# Autodesk Inventor assembly: testframe
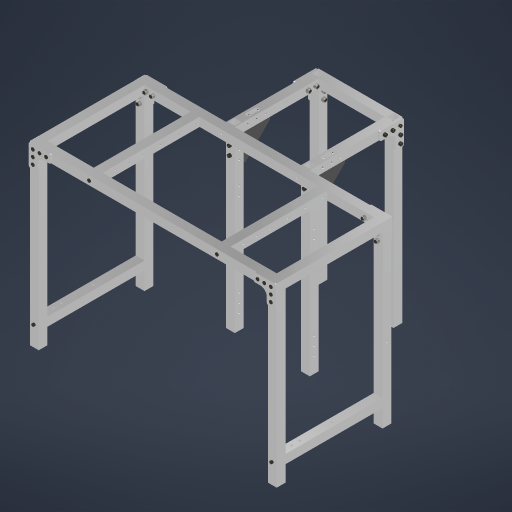
[picture p0: Inventor's stored thumbnail of the model, 512x512]
Saved by Autodesk Inventor 2024.2 (Build 282272000, 272)
## iProperties
Created: 2024-07-23
Part Number: testframe
Document SubType Name: Assembly
Designer: bryan
Mass: 7374.18 g
Surface Area: 16423.9 cm^2
Volume: 2648.19 cm^3
Density: 2.78461 g/cm^3
Author: bryan
## Documents named in this file (28)
- C:\Users\bobsb\OneDrive\Documents\GitHub\1622-2024-Summer-CAD-A-Thon\Structure\STRU_000_StructureAssembly.iam
- C:\Users\bobsb\OneDrive\Documents\GitHub\1622-2024-Summer-CAD-A-Thon\Structure\STRU_001_BilletBlock.ipt
- C:\Users\bobsb\OneDrive\Documents\GitHub\1622-2024-Summer-CAD-A-Thon\Structure\STRU_002_BilletPole_20.56in_Angled.ipt
- C:\Users\bobsb\OneDrive\Documents\GitHub\1622-2024-Summer-CAD-A-Thon\Structure\STRU_003_BilletPole_28in_Angled.ipt
- C:\Users\bobsb\OneDrive\Documents\GitHub\1622-2024-Summer-CAD-A-Thon\Structure\STRU_004_DoubleBillet_90_2.25in.ipt
- C:\Users\bobsb\OneDrive\Documents\GitHub\1622-2024-Summer-CAD-A-Thon\Structure\STRU_007_BilletPole_11in.ipt
- C:\Users\bobsb\OneDrive\Documents\GitHub\1622-2024-Summer-CAD-A-Thon\Structure\STRU_003_BilletPole_28in_Angled_Unique.ipt
- C:\Users\bobsb\OneDrive\Documents\GitHub\1622-2024-Summer-CAD-A-Thon\COTS Library\Fasteners\Bolts\Socket-Head\10-32\COTS_90044A120_Black-Oxide Alloy Steel Socket Head Screw.ipt
- C:\Users\bobsb\OneDrive\Documents\GitHub\1622-2024-Summer-CAD-A-Thon\COTS Library\Fasteners\Bolts\Socket-Head\0.25-20\COTS_90044A123_Black-Oxide Alloy Steel Socket Head Screw.ipt
- C:\Users\bobsb\OneDrive\Documents\GitHub\1622-2024-Summer-CAD-A-Thon\COTS Library\Fasteners\Nuts\COTS_95615A120_Medium-Strength Steel Nylon-Insert Locknut.ipt
- C:\Users\bobsb\OneDrive\Documents\GitHub\1622-2024-Summer-CAD-A-Thon\Structure\STRU_009_FrameBracket_90.ipt
- C:\Users\bobsb\OneDrive\Documents\GitHub\1622-2024-Summer-CAD-A-Thon\Structure\STRU_006_BilletPole_SwerveOffset.ipt
- C:\Users\bobsb\OneDrive\Documents\GitHub\1622-2024-Summer-CAD-A-Thon\Structure\STRU_012_BilletPoleMiddle.ipt
- C:\Users\bobsb\OneDrive\Documents\GitHub\1622-2024-Summer-CAD-A-Thon\Structure\STRU_012_BilletPoleMiddle_Unique.ipt
- C:\Users\bobsb\OneDrive\Documents\GitHub\1622-2024-Summer-CAD-A-Thon\Structure\STRU_014_BilletPole_9in_Angled.ipt
- C:\Users\bobsb\OneDrive\Documents\GitHub\1622-2024-Summer-CAD-A-Thon\Structure\STRU_015_BilletPole_9in.ipt
- C:\Users\bobsb\OneDrive\Documents\GitHub\1622-2024-Summer-CAD-A-Thon\Structure\STRU_016_FrameBracket2_90.ipt
- C:\Users\bobsb\OneDrive\Documents\GitHub\1622-2024-Summer-CAD-A-Thon\Structure\STRU_017_AngleBracket_90_Plastic.ipt
- C:\Users\bobsb\OneDrive\Documents\GitHub\1622-2024-Summer-CAD-A-Thon\COTS Library\Fasteners\Bolts\Socket-Head\0.25-20\COTS_91251A539_Black-Oxide Alloy Steel Socket Head Screw (1).ipt
- C:\Users\bobsb\OneDrive\Documents\GitHub\1622-2024-Summer-CAD-A-Thon\COTS Library\Fasteners\Nuts\COTS_95462A029_Medium-Strength Steel Hex Nut (2).ipt
- C:\Users\bobsb\OneDrive\Documents\GitHub\1622-2024-Summer-CAD-A-Thon\Structure\STRU_019_RubberWasher.ipt
- C:\Users\bobsb\OneDrive\Documents\GitHub\1622-2024-Summer-CAD-A-Thon\Structure\STRU_023_Kenji_11in.ipt
- C:\Users\bobsb\OneDrive\Documents\GitHub\1622-2024-Summer-CAD-A-Thon\Structure\STRU_024_BilletBlock2.ipt
- C:\Users\bobsb\OneDrive\Documents\GitHub\1622-2024-Summer-CAD-A-Thon\COTS Library\Fasteners\Bolts\Socket-Head\0.25-20\COTS_90357A018_Ultra-Low-Profile Socket Head Screw.ipt
- C:\Users\bobsb\OneDrive\Documents\GitHub\1622-2024-Summer-CAD-A-Thon\COTS Library\Fasteners\Bolts\Socket-Head\0.25-20\COTS_90357A021_Ultra-Low-Profile Socket Head Screw.ipt
- C:\Users\bobsb\OneDrive\Documents\GitHub\1622-2024-Summer-CAD-A-Thon\COTS Library\Fasteners\Bolts\Socket-Head\10-32\COTS_91251A352_Black-Oxide Alloy Steel Socket Head.ipt
- C:\Users\bobsb\OneDrive\Documents\GitHub\1622-2024-Summer-CAD-A-Thon\Structure\STRU_026_Bryan_11in.ipt
- C:\Users\bobsb\OneDrive\Documents\GitHub\1622-2024-Summer-CAD-A-Thon\Structure\STRU_000_StructureAssembly\AIP\FEA\err5tqxb5.fres
## Components (137 placed, 26 different names)
1. STRU_001_BilletBlock:2 — Mate:16, Mate:17, Flush:2
2. STRU_002_BilletPole_20.56in_Angled:1 — Mate:1, Mate:4, Mate:5, Mate:41, Mate:53, Mate:54, Flush:10, Mate:91, Mate:92, Mate:127, Mate:147, Mate:148, Mate:470, Mate:471, Flush:63, Mate:527, Mate:528
3. STRU_004_DoubleBillet_90_2.25in:1 — Mate:1, Mate:4, Mate:5, Mate:34, Mate:56, Mate:58, Mate:125, Mate:126
4. STRU_002_BilletPole_20.56in_Angled:2 — Mate:13, Mate:14, Mate:15, Mate:16, Mate:17, Flush:2, Mate:40, Mate:85, Mate:86, Mate:123, Mate:124, Mate:145, Mate:146, Mate:477, Mate:478, Mate:531, Mate:532, Flush:71
5. STRU_004_DoubleBillet_90_2.25in:2 — Mate:13, Mate:14, Mate:15, Mate:36, Mate:57, Mate:100, Mate:121, Mate:122
6. STRU_001_BilletBlock:3 — Mate:185, Mate:186, Flush:26
7. STRU_001_BilletBlock:4 — Mate:180, Mate:181, Flush:25
8. STRU_003_BilletPole_28in_Angled:2 — Mate:47, Flush:8, Flush:9, Mate:55, Mate:118, Mate:130, Mate:153, Mate:154, Mate:155, Mate:156, Mate:178, Mate:182, Mate:484, Mate:485, Mate:486, Mate:490, Flush:68, Mate:491, Mate:492, Mate:493, Mate:541, Flush:73, Mate:542, Mate:543, Mate:544, Mate:545, Flush:74, Mate:548
9. STRU_004_DoubleBillet_90_2.25in:3 — Mate:128, Mate:129, Mate:184
10. STRU_004_DoubleBillet_90_2.25in:4 — Mate:119, Mate:120, Mate:179
11. STRU_001_BilletBlock:5 — Mate:34, Mate:41, Mate:50, Mate:51, Flush:65
12. STRU_001_BilletBlock:8 — Mate:36, Mate:40, Mate:42, Mate:43
13. STRU_007_BilletPole_11in:1 — Flush:9, Mate:50, Mate:51, Mate:55, Mate:59, Mate:537
14. STRU_007_BilletPole_11in:2 — Mate:42, Mate:43, Mate:47, Flush:8, Mate:124
15. STRU_001_BilletBlock:9 — Mate:53, Mate:54, Flush:10
16. STRU_003_BilletPole_28in_Angled_Unique:1 — Mate:56, Mate:57, Mate:58, Mate:59, Mate:83, Mate:84, Mate:93, Mate:94, Mate:98, Mate:149, Mate:150, Mate:151, Mate:152, Mate:159, Mate:160, Mate:164, Mate:165, Flush:28, Mate:221, Flush:29, Mate:223, Flush:68, Mate:559
17. COTS_90044A123_Black-Oxide Alloy Steel Socket Head Screw:6 — Mate:84, Mate:108, Flush:12
18. COTS_90044A123_Black-Oxide Alloy Steel Socket Head Screw:7 — Mate:85, Mate:106, Mate:134, Flush:12, Flush:13, Flush:14
19. COTS_90044A123_Black-Oxide Alloy Steel Socket Head Screw:8 — Mate:83, Mate:107, Flush:13
20. COTS_90044A123_Black-Oxide Alloy Steel Socket Head Screw:9 — Mate:86, Mate:105, Flush:14
21. COTS_90044A123_Black-Oxide Alloy Steel Socket Head Screw:14 — Mate:93, Mate:115, Flush:16
22. COTS_90044A123_Black-Oxide Alloy Steel Socket Head Screw:15 — Mate:92, Mate:114, Flush:17
23. COTS_90044A123_Black-Oxide Alloy Steel Socket Head Screw:16 — Mate:91, Mate:113, Mate:136, Flush:15, Flush:17
24. COTS_90044A123_Black-Oxide Alloy Steel Socket Head Screw:17 — Mate:94, Mate:116, Flush:15, Flush:16
25. COTS_90044A120_Black-Oxide Alloy Steel Socket Head Screw:6 — Mate:100, Mate:135
26. COTS_90044A120_Black-Oxide Alloy Steel Socket Head Screw:7 — Mate:98, Mate:137
27. COTS_95615A120_Medium-Strength Steel Nylon-Insert Locknut:1 — Mate:154, Mate:522
28. COTS_95615A120_Medium-Strength Steel Nylon-Insert Locknut:2 — Mate:153, Mate:521
29. COTS_95615A120_Medium-Strength Steel Nylon-Insert Locknut:3 — Mate:194, Mate:519
30. COTS_95615A120_Medium-Strength Steel Nylon-Insert Locknut:4 — Mate:195, Mate:520
31. COTS_95615A120_Medium-Strength Steel Nylon-Insert Locknut:5 — Mate:107, Mate:152
32. COTS_95615A120_Medium-Strength Steel Nylon-Insert Locknut:6 — Mate:108, Mate:151
33. COTS_95615A120_Medium-Strength Steel Nylon-Insert Locknut:7 — Mate:105, Mate:145
34. COTS_95615A120_Medium-Strength Steel Nylon-Insert Locknut:8 — Mate:106, Mate:146
35. COTS_95615A120_Medium-Strength Steel Nylon-Insert Locknut:9 — Mate:155, Mate:514
36. COTS_95615A120_Medium-Strength Steel Nylon-Insert Locknut:10 — Mate:156, Mate:515
37. COTS_95615A120_Medium-Strength Steel Nylon-Insert Locknut:11 — Mate:189, Mate:513
38. COTS_95615A120_Medium-Strength Steel Nylon-Insert Locknut:12 — Mate:190, Mate:512
39. COTS_95615A120_Medium-Strength Steel Nylon-Insert Locknut:13 — Mate:114, Mate:147
40. COTS_95615A120_Medium-Strength Steel Nylon-Insert Locknut:14 — Mate:113, Mate:148
41. COTS_95615A120_Medium-Strength Steel Nylon-Insert Locknut:15 — Mate:115, Mate:149
42. COTS_95615A120_Medium-Strength Steel Nylon-Insert Locknut:16 — Mate:116, Mate:150
43. STRU_009_FrameBracket_90:1 — Mate:118, Mate:119, Mate:120, Mate:177, Mate:497, Mate:498, Mate:499, Mate:500, Mate:501, Mate:502, Mate:503, Mate:516, Mate:517, Mate:518
44. STRU_009_FrameBracket_90:2 — Mate:125, Mate:126, Mate:127, Mate:136, Mate:137
45. STRU_009_FrameBracket_90:3 — Mate:121, Mate:122, Mate:123, Mate:134, Mate:135
46. STRU_009_FrameBracket_90:4 — Mate:128, Mate:129, Mate:130, Mate:183, Mate:504, Mate:505, Mate:506, Mate:507, Mate:508, Mate:509, Mate:510, Mate:511, Mate:523, Mate:524
47. STRU_001_BilletBlock:11 — Mate:159, Mate:165
48. STRU_001_BilletBlock:12 — Mate:160, Mate:164, Flush:66
49. STRU_006_BilletPole_SwerveOffset:1 — Mate:177, Mate:178, Mate:179, Mate:180, Mate:181, Flush:25, Mate:194, Mate:195, Mate:487, Mate:489, Mate:494, Mate:529, Mate:530, Mate:533
50. STRU_006_BilletPole_SwerveOffset:2 — Mate:182, Mate:183, Mate:184, Mate:185, Mate:186, Flush:26, Mate:189, Mate:190, Mate:475, Mate:488, Mate:495, Mate:525, Mate:526
51. STRU_012_BilletPoleMiddle:6 — Flush:28, Mate:221, Mate:228, Mate:229, Flush:30, Mate:255, Flush:49, Mate:318, Mate:389, Mate:390, Mate:418, Mate:419, Mate:559
52. STRU_012_BilletPoleMiddle:5 — Flush:29, Mate:223, Mate:230, Mate:231, Flush:31, Mate:253, Flush:48, Mate:319, Mate:391, Mate:392, Mate:416, Mate:417
53. STRU_001_BilletBlock:14 — Mate:228, Mate:229, Flush:30
54. STRU_001_BilletBlock:15 — Mate:230, Mate:231, Flush:31
55. STRU_001_BilletBlock:16 — Mate:267, Mate:268, Flush:54
56. STRU_001_BilletBlock:17 — Mate:269, Mate:270, Flush:55
57. STRU_014_BilletPole_9in_Angled:1 — Mate:255, Flush:49, Mate:311, Mate:317, Mate:333, Mate:334, Mate:335, Mate:336, Mate:549, Mate:551, Mate:552, Mate:557, Mate:558
58. STRU_014_BilletPole_9in_Angled:2 — Mate:253, Flush:48, Mate:291, Mate:320, Mate:337, Mate:338, Mate:339, Mate:340, Mate:550, Mate:553, Mate:554, Mate:555, Flush:75, Mate:556
59. STRU_015_BilletPole_9in:1 — Mate:257, Mate:258, Mate:259, Mate:260, Flush:52, Flush:53, Flush:75
60. STRU_001_BilletBlock:18 — Mate:259, Mate:260, Flush:52, Mate:266, Mate:271, Mate:275
61. STRU_001_BilletBlock:19 — Mate:257, Mate:258, Flush:53, Mate:265, Mate:272, Mate:276
62. STRU_012_BilletPoleMiddle_Unique:1 — Mate:265, Mate:267, Mate:268, Flush:54, Mate:272, Mate:277, Mate:278, Mate:279, Mate:304, Mate:316
63. STRU_012_BilletPoleMiddle_Unique:2 — Mate:266, Mate:269, Mate:270, Flush:55, Mate:271, Mate:281, Mate:282, Mate:283, Mate:295, Mate:299
64. COTS_90044A120_Black-Oxide Alloy Steel Socket Head Screw:13 — Mate:275, Mate:284
65. COTS_90044A120_Black-Oxide Alloy Steel Socket Head Screw:14 — Mate:276, Mate:280
66. STRU_016_FrameBracket2_90:1 — Mate:277, Mate:278, Mate:279, Mate:280, Mate:302, Mate:303, Mate:306, Mate:307, Mate:310, Mate:312, Mate:314, Mate:315, Mate:558
67. STRU_016_FrameBracket2_90:2 — Mate:281, Mate:282, Mate:283, Mate:284, Mate:286, Mate:288, Mate:290, Mate:292, Mate:294, Mate:296, Mate:298, Mate:300, Mate:555
68. COTS_90044A123_Black-Oxide Alloy Steel Socket Head Screw:18 — Mate:286, Mate:288, Mate:553
69. COTS_95615A120_Medium-Strength Steel Nylon-Insert Locknut:17 — Mate:556
70. COTS_90044A123_Black-Oxide Alloy Steel Socket Head Screw:19 — Mate:290, Mate:292, Mate:554
71. COTS_95615A120_Medium-Strength Steel Nylon-Insert Locknut:18 — Mate:291
72. COTS_90044A123_Black-Oxide Alloy Steel Socket Head Screw:20 — Mate:294, Mate:296
73. COTS_95615A120_Medium-Strength Steel Nylon-Insert Locknut:19 — Mate:295
74. COTS_90044A123_Black-Oxide Alloy Steel Socket Head Screw:21 — Mate:298, Mate:300
75. COTS_95615A120_Medium-Strength Steel Nylon-Insert Locknut:20 — Mate:299
76. COTS_90044A123_Black-Oxide Alloy Steel Socket Head Screw:22 — Mate:302, Mate:303
77. COTS_95615A120_Medium-Strength Steel Nylon-Insert Locknut:21 — Mate:304
78. COTS_90044A123_Black-Oxide Alloy Steel Socket Head Screw:23 — Mate:306, Mate:307, Mate:551
79. COTS_95615A120_Medium-Strength Steel Nylon-Insert Locknut:22 — Mate:557
80. COTS_90044A123_Black-Oxide Alloy Steel Socket Head Screw:24 — Mate:310, Mate:312, Mate:552
81. COTS_95615A120_Medium-Strength Steel Nylon-Insert Locknut:23 — Mate:311
82. COTS_90044A123_Black-Oxide Alloy Steel Socket Head Screw:25 — Mate:314, Mate:315
83. COTS_95615A120_Medium-Strength Steel Nylon-Insert Locknut:24 — Mate:316
84. STRU_017_AngleBracket_90_Plastic:1 — Mate:317, Mate:318, Mate:453, Mate:454, Mate:458, Mate:462, Mate:463, Mate:467, Mate:549
85. STRU_017_AngleBracket_90_Plastic:2 — Mate:319, Mate:320, Mate:434, Mate:435, Mate:440, Mate:444, Mate:445, Mate:449, Mate:550
86. COTS_91251A539_Black-Oxide Alloy Steel Socket Head Screw (1):1 — Mate:337, Mate:340, Mate:439
87. COTS_91251A539_Black-Oxide Alloy Steel Socket Head Screw (1):2 — Mate:338, Mate:339, Mate:432, Mate:433
88. COTS_91251A539_Black-Oxide Alloy Steel Socket Head Screw (1):4 — Mate:333, Mate:334, Mate:457
89. COTS_91251A539_Black-Oxide Alloy Steel Socket Head Screw (1):5 — Mate:335, Mate:336, Mate:452
90. COTS_90044A123_Black-Oxide Alloy Steel Socket Head Screw:27 — Mate:390, Mate:419, Mate:461
91. COTS_90044A123_Black-Oxide Alloy Steel Socket Head Screw:28 — Mate:389, Mate:418, Mate:466
92. COTS_90044A123_Black-Oxide Alloy Steel Socket Head Screw:29 — Mate:392, Mate:417, Mate:448
93. COTS_90044A123_Black-Oxide Alloy Steel Socket Head Screw:30 — Mate:391, Mate:416, Mate:442, Mate:443
94. COTS_95462A029_Medium-Strength Steel Hex Nut (2):1 — Mate:432, Mate:436
95. STRU_019_RubberWasher:1 — Mate:433, Mate:434, Mate:435, Mate:436, Flush:59
96. COTS_95462A029_Medium-Strength Steel Hex Nut (2):2 — Mate:438, Mate:439
97. STRU_019_RubberWasher:2 — Mate:438, Flush:59, Mate:440
98. COTS_95462A029_Medium-Strength Steel Hex Nut (2):3 — Mate:442
99. STRU_019_RubberWasher:3 — Mate:443, Mate:444, Mate:445, Flush:60
100. COTS_95462A029_Medium-Strength Steel Hex Nut (2):4 — Mate:447, Mate:448
101. STRU_019_RubberWasher:4 — Mate:447, Mate:449, Flush:60
102. COTS_95462A029_Medium-Strength Steel Hex Nut (2):5 — Mate:452
103. STRU_019_RubberWasher:5 — Mate:453, Mate:454, Flush:61
104. COTS_95462A029_Medium-Strength Steel Hex Nut (2):6 — Mate:457
105. STRU_019_RubberWasher:6 — Mate:458, Flush:61
106. COTS_95462A029_Medium-Strength Steel Hex Nut (2):7 — Mate:461
107. STRU_019_RubberWasher:7 — Mate:462, Mate:463, Flush:62
108. COTS_95462A029_Medium-Strength Steel Hex Nut (2):8 — Mate:466
109. STRU_019_RubberWasher:8 — Mate:467, Flush:62
110. STRU_023_Kenji_11in:1 — Mate:472, Mate:473, Flush:63, Mate:475
111. STRU_023_Kenji_11in:2 — Mate:533, Flush:71, Mate:534
112. STRU_001_BilletBlock:22 — Mate:470, Mate:471, Mate:472, Mate:473
113. STRU_001_BilletBlock:23 — Mate:477, Mate:478, Mate:534
114. STRU_024_BilletBlock2:1 — Mate:484, Mate:490, Flush:65, Mate:537
115. STRU_024_BilletBlock2:2 — Mate:487, Flush:69, Mate:492
116. STRU_024_BilletBlock2:3 — Mate:488, Mate:495, Flush:70
117. STRU_024_BilletBlock2:4 — Mate:489, Mate:494, Flush:70
118. STRU_024_BilletBlock2:5 — Mate:486, Flush:67, Flush:69, Mate:491, Mate:539, Mate:540
119. STRU_024_BilletBlock2:6 — Mate:485, Flush:66, Flush:67, Mate:493, Mate:546, Mate:547
120. COTS_90357A018_Ultra-Low-Profile Socket Head Screw:1 — Mate:499, Mate:500, Mate:521
121. COTS_90357A021_Ultra-Low-Profile Socket Head Screw:1 — Mate:497, Mate:498
122. COTS_90357A018_Ultra-Low-Profile Socket Head Screw:2 — Mate:501, Mate:516, Mate:522
123. COTS_90357A018_Ultra-Low-Profile Socket Head Screw:3 — Mate:502, Mate:518, Mate:519
124. COTS_90357A018_Ultra-Low-Profile Socket Head Screw:4 — Mate:503, Mate:517, Mate:520
125. COTS_90357A018_Ultra-Low-Profile Socket Head Screw:5 — Mate:504, Mate:508, Mate:514
126. COTS_90357A018_Ultra-Low-Profile Socket Head Screw:6 — Mate:505, Mate:509, Mate:515
127. COTS_90357A018_Ultra-Low-Profile Socket Head Screw:7 — Mate:506, Mate:510, Mate:513
128. COTS_90357A018_Ultra-Low-Profile Socket Head Screw:8 — Mate:507, Mate:511, Mate:512
129. COTS_90357A021_Ultra-Low-Profile Socket Head Screw:2 — Mate:523, Mate:524
130. COTS_91251A352_Black-Oxide Alloy Steel Socket Head:1 — Mate:525, Mate:526
131. COTS_91251A352_Black-Oxide Alloy Steel Socket Head:2 — Mate:527, Mate:528
132. COTS_91251A352_Black-Oxide Alloy Steel Socket Head:3 — Mate:529, Mate:530
133. COTS_91251A352_Black-Oxide Alloy Steel Socket Head:4 — Mate:531, Mate:532
134. STRU_026_Bryan_11in:2 — Mate:539, Mate:540, Mate:541, Flush:73
135. COTS_90357A021_Ultra-Low-Profile Socket Head Screw:3 — Mate:542, Mate:543
136. COTS_90357A021_Ultra-Low-Profile Socket Head Screw:4 — Mate:544, Mate:545
137. STRU_026_Bryan_11in:3 — Mate:546, Mate:547, Flush:74, Mate:548
## Relationships (327: Mate 290, Flush 37)
- Mate:1: STRU_002_BilletPole_20.56in_Angled:1 ↔ STRU_004_DoubleBillet_90_2.25in:1
- Mate:4: STRU_002_BilletPole_20.56in_Angled:1 ↔ STRU_004_DoubleBillet_90_2.25in:1
- Mate:5: STRU_002_BilletPole_20.56in_Angled:1 ↔ STRU_004_DoubleBillet_90_2.25in:1
- Mate:13: STRU_002_BilletPole_20.56in_Angled:2 ↔ STRU_004_DoubleBillet_90_2.25in:2
- Mate:14: STRU_002_BilletPole_20.56in_Angled:2 ↔ STRU_004_DoubleBillet_90_2.25in:2
- Mate:15: STRU_002_BilletPole_20.56in_Angled:2 ↔ STRU_004_DoubleBillet_90_2.25in:2
- Mate:16: STRU_001_BilletBlock:2 ↔ STRU_002_BilletPole_20.56in_Angled:2
- Mate:17: STRU_001_BilletBlock:2 ↔ STRU_002_BilletPole_20.56in_Angled:2
- Flush:2: STRU_001_BilletBlock:2 ↔ STRU_002_BilletPole_20.56in_Angled:2
- [Mate]: STRU_003_BilletPole_28in_Angled:2 ↔ STRU_004_DoubleBillet_90_2.25in:3
- [Mate]: STRU_003_BilletPole_28in_Angled:2 ↔ STRU_004_DoubleBillet_90_2.25in:3
- [Mate]: STRU_003_BilletPole_28in_Angled:2 ↔ STRU_004_DoubleBillet_90_2.25in:3
- [Mate]: STRU_003_BilletPole_28in_Angled:2 ↔ STRU_004_DoubleBillet_90_2.25in:4
- [Mate]: STRU_003_BilletPole_28in_Angled:2 ↔ STRU_004_DoubleBillet_90_2.25in:4
- [Mate]: STRU_003_BilletPole_28in_Angled:2 ↔ STRU_004_DoubleBillet_90_2.25in:4
- Mate:34: STRU_004_DoubleBillet_90_2.25in:1 ↔ STRU_001_BilletBlock:5
- Mate:36: STRU_004_DoubleBillet_90_2.25in:2 ↔ STRU_001_BilletBlock:8
- Mate:40: STRU_002_BilletPole_20.56in_Angled:2 ↔ STRU_001_BilletBlock:8
- Mate:41: STRU_002_BilletPole_20.56in_Angled:1 ↔ STRU_001_BilletBlock:5
- Mate:42: STRU_001_BilletBlock:8 ↔ STRU_007_BilletPole_11in:2
- Mate:43: STRU_001_BilletBlock:8 ↔ STRU_007_BilletPole_11in:2
- Mate:47: STRU_003_BilletPole_28in_Angled:2 ↔ STRU_007_BilletPole_11in:2
- Flush:8: STRU_003_BilletPole_28in_Angled:2 ↔ STRU_007_BilletPole_11in:2
- Flush:9: STRU_003_BilletPole_28in_Angled:2 ↔ STRU_007_BilletPole_11in:1
- Mate:50: STRU_001_BilletBlock:5 ↔ STRU_007_BilletPole_11in:1
- Mate:51: STRU_001_BilletBlock:5 ↔ STRU_007_BilletPole_11in:1
- Mate:53: STRU_002_BilletPole_20.56in_Angled:1 ↔ STRU_001_BilletBlock:9
- Mate:54: STRU_002_BilletPole_20.56in_Angled:1 ↔ STRU_001_BilletBlock:9
- Flush:10: STRU_002_BilletPole_20.56in_Angled:1 ↔ STRU_001_BilletBlock:9
- Mate:55: STRU_003_BilletPole_28in_Angled:2 ↔ STRU_007_BilletPole_11in:1
- Mate:56: STRU_004_DoubleBillet_90_2.25in:1 ↔ STRU_003_BilletPole_28in_Angled_Unique:1
- Mate:57: STRU_004_DoubleBillet_90_2.25in:2 ↔ STRU_003_BilletPole_28in_Angled_Unique:1
- Mate:58: STRU_004_DoubleBillet_90_2.25in:1 ↔ STRU_003_BilletPole_28in_Angled_Unique:1
- Mate:59: STRU_007_BilletPole_11in:1 ↔ STRU_003_BilletPole_28in_Angled_Unique:1
- Mate:83: STRU_003_BilletPole_28in_Angled_Unique:1 ↔ COTS_90044A123_Black-Oxide Alloy Steel Socket Head Screw:8
- Mate:84: STRU_003_BilletPole_28in_Angled_Unique:1 ↔ COTS_90044A123_Black-Oxide Alloy Steel Socket Head Screw:6
- Mate:85: STRU_002_BilletPole_20.56in_Angled:2 ↔ COTS_90044A123_Black-Oxide Alloy Steel Socket Head Screw:7
- Mate:86: STRU_002_BilletPole_20.56in_Angled:2 ↔ COTS_90044A123_Black-Oxide Alloy Steel Socket Head Screw:9
- Mate:91: STRU_002_BilletPole_20.56in_Angled:1 ↔ COTS_90044A123_Black-Oxide Alloy Steel Socket Head Screw:16
- Mate:92: STRU_002_BilletPole_20.56in_Angled:1 ↔ COTS_90044A123_Black-Oxide Alloy Steel Socket Head Screw:15
- Mate:93: STRU_003_BilletPole_28in_Angled_Unique:1 ↔ COTS_90044A123_Black-Oxide Alloy Steel Socket Head Screw:14
- Mate:94: STRU_003_BilletPole_28in_Angled_Unique:1 ↔ COTS_90044A123_Black-Oxide Alloy Steel Socket Head Screw:17
- Mate:98: STRU_003_BilletPole_28in_Angled_Unique:1 ↔ COTS_90044A120_Black-Oxide Alloy Steel Socket Head Screw:7
- Mate:100: STRU_004_DoubleBillet_90_2.25in:2 ↔ COTS_90044A120_Black-Oxide Alloy Steel Socket Head Screw:6
- Mate:105: COTS_90044A123_Black-Oxide Alloy Steel Socket Head Screw:9 ↔ COTS_95615A120_Medium-Strength Steel Nylon-Insert Locknut:7
- Mate:106: COTS_90044A123_Black-Oxide Alloy Steel Socket Head Screw:7 ↔ COTS_95615A120_Medium-Strength Steel Nylon-Insert Locknut:8
- Mate:107: COTS_90044A123_Black-Oxide Alloy Steel Socket Head Screw:8 ↔ COTS_95615A120_Medium-Strength Steel Nylon-Insert Locknut:5
- Mate:108: COTS_90044A123_Black-Oxide Alloy Steel Socket Head Screw:6 ↔ COTS_95615A120_Medium-Strength Steel Nylon-Insert Locknut:6
- Mate:113: COTS_90044A123_Black-Oxide Alloy Steel Socket Head Screw:16 ↔ COTS_95615A120_Medium-Strength Steel Nylon-Insert Locknut:14
- Mate:114: COTS_90044A123_Black-Oxide Alloy Steel Socket Head Screw:15 ↔ COTS_95615A120_Medium-Strength Steel Nylon-Insert Locknut:13
- Mate:115: COTS_90044A123_Black-Oxide Alloy Steel Socket Head Screw:14 ↔ COTS_95615A120_Medium-Strength Steel Nylon-Insert Locknut:15
- Mate:116: COTS_90044A123_Black-Oxide Alloy Steel Socket Head Screw:17 ↔ COTS_95615A120_Medium-Strength Steel Nylon-Insert Locknut:16
- Mate:118: STRU_003_BilletPole_28in_Angled:2 ↔ STRU_009_FrameBracket_90:1
- Mate:119: STRU_004_DoubleBillet_90_2.25in:4 ↔ STRU_009_FrameBracket_90:1
- Mate:120: STRU_004_DoubleBillet_90_2.25in:4 ↔ STRU_009_FrameBracket_90:1
- Mate:121: STRU_004_DoubleBillet_90_2.25in:2 ↔ STRU_009_FrameBracket_90:3
- Mate:122: STRU_004_DoubleBillet_90_2.25in:2 ↔ STRU_009_FrameBracket_90:3
- Mate:123: STRU_002_BilletPole_20.56in_Angled:2 ↔ STRU_009_FrameBracket_90:3
- Mate:124: STRU_002_BilletPole_20.56in_Angled:2 ↔ STRU_007_BilletPole_11in:2
- Mate:125: STRU_004_DoubleBillet_90_2.25in:1 ↔ STRU_009_FrameBracket_90:2
- Mate:126: STRU_004_DoubleBillet_90_2.25in:1 ↔ STRU_009_FrameBracket_90:2
- Mate:127: STRU_002_BilletPole_20.56in_Angled:1 ↔ STRU_009_FrameBracket_90:2
- Mate:128: STRU_004_DoubleBillet_90_2.25in:3 ↔ STRU_009_FrameBracket_90:4
- Mate:129: STRU_004_DoubleBillet_90_2.25in:3 ↔ STRU_009_FrameBracket_90:4
- Mate:130: STRU_003_BilletPole_28in_Angled:2 ↔ STRU_009_FrameBracket_90:4
- Mate:134: COTS_90044A123_Black-Oxide Alloy Steel Socket Head Screw:7 ↔ STRU_009_FrameBracket_90:3
- Flush:12: COTS_90044A123_Black-Oxide Alloy Steel Socket Head Screw:6 ↔ COTS_90044A123_Black-Oxide Alloy Steel Socket Head Screw:7
- Mate:135: COTS_90044A120_Black-Oxide Alloy Steel Socket Head Screw:6 ↔ STRU_009_FrameBracket_90:3
- Flush:13: COTS_90044A123_Black-Oxide Alloy Steel Socket Head Screw:7 ↔ COTS_90044A123_Black-Oxide Alloy Steel Socket Head Screw:8
- Flush:14: COTS_90044A123_Black-Oxide Alloy Steel Socket Head Screw:7 ↔ COTS_90044A123_Black-Oxide Alloy Steel Socket Head Screw:9
- Mate:136: COTS_90044A123_Black-Oxide Alloy Steel Socket Head Screw:16 ↔ STRU_009_FrameBracket_90:2
- Mate:137: COTS_90044A120_Black-Oxide Alloy Steel Socket Head Screw:7 ↔ STRU_009_FrameBracket_90:2
- Flush:15: COTS_90044A123_Black-Oxide Alloy Steel Socket Head Screw:16 ↔ COTS_90044A123_Black-Oxide Alloy Steel Socket Head Screw:17
- Flush:16: COTS_90044A123_Black-Oxide Alloy Steel Socket Head Screw:14 ↔ COTS_90044A123_Black-Oxide Alloy Steel Socket Head Screw:17
- Flush:17: COTS_90044A123_Black-Oxide Alloy Steel Socket Head Screw:15 ↔ COTS_90044A123_Black-Oxide Alloy Steel Socket Head Screw:16
- Mate:145: STRU_002_BilletPole_20.56in_Angled:2 ↔ COTS_95615A120_Medium-Strength Steel Nylon-Insert Locknut:7
- Mate:146: STRU_002_BilletPole_20.56in_Angled:2 ↔ COTS_95615A120_Medium-Strength Steel Nylon-Insert Locknut:8
- Mate:147: STRU_002_BilletPole_20.56in_Angled:1 ↔ COTS_95615A120_Medium-Strength Steel Nylon-Insert Locknut:13
- Mate:148: STRU_002_BilletPole_20.56in_Angled:1 ↔ COTS_95615A120_Medium-Strength Steel Nylon-Insert Locknut:14
- Mate:149: STRU_003_BilletPole_28in_Angled_Unique:1 ↔ COTS_95615A120_Medium-Strength Steel Nylon-Insert Locknut:15
- Mate:150: STRU_003_BilletPole_28in_Angled_Unique:1 ↔ COTS_95615A120_Medium-Strength Steel Nylon-Insert Locknut:16
- Mate:151: STRU_003_BilletPole_28in_Angled_Unique:1 ↔ COTS_95615A120_Medium-Strength Steel Nylon-Insert Locknut:6
- Mate:152: STRU_003_BilletPole_28in_Angled_Unique:1 ↔ COTS_95615A120_Medium-Strength Steel Nylon-Insert Locknut:5
- Mate:153: STRU_003_BilletPole_28in_Angled:2 ↔ COTS_95615A120_Medium-Strength Steel Nylon-Insert Locknut:2
- Mate:154: STRU_003_BilletPole_28in_Angled:2 ↔ COTS_95615A120_Medium-Strength Steel Nylon-Insert Locknut:1
- Mate:155: STRU_003_BilletPole_28in_Angled:2 ↔ COTS_95615A120_Medium-Strength Steel Nylon-Insert Locknut:9
- Mate:156: STRU_003_BilletPole_28in_Angled:2 ↔ COTS_95615A120_Medium-Strength Steel Nylon-Insert Locknut:10
- Mate:159: STRU_003_BilletPole_28in_Angled_Unique:1 ↔ STRU_001_BilletBlock:11
- Mate:160: STRU_003_BilletPole_28in_Angled_Unique:1 ↔ STRU_001_BilletBlock:12
- Mate:164: STRU_003_BilletPole_28in_Angled_Unique:1 ↔ STRU_001_BilletBlock:12
- Mate:165: STRU_003_BilletPole_28in_Angled_Unique:1 ↔ STRU_001_BilletBlock:11
- Mate:177: STRU_009_FrameBracket_90:1 ↔ STRU_006_BilletPole_SwerveOffset:1
- Mate:178: STRU_003_BilletPole_28in_Angled:2 ↔ STRU_006_BilletPole_SwerveOffset:1
- Mate:179: STRU_004_DoubleBillet_90_2.25in:4 ↔ STRU_006_BilletPole_SwerveOffset:1
- Mate:180: STRU_001_BilletBlock:4 ↔ STRU_006_BilletPole_SwerveOffset:1
- Mate:181: STRU_001_BilletBlock:4 ↔ STRU_006_BilletPole_SwerveOffset:1
- Flush:25: STRU_001_BilletBlock:4 ↔ STRU_006_BilletPole_SwerveOffset:1
- Mate:182: STRU_003_BilletPole_28in_Angled:2 ↔ STRU_006_BilletPole_SwerveOffset:2
- Mate:183: STRU_009_FrameBracket_90:4 ↔ STRU_006_BilletPole_SwerveOffset:2
- Mate:184: STRU_004_DoubleBillet_90_2.25in:3 ↔ STRU_006_BilletPole_SwerveOffset:2
- Mate:185: STRU_001_BilletBlock:3 ↔ STRU_006_BilletPole_SwerveOffset:2
- Mate:186: STRU_001_BilletBlock:3 ↔ STRU_006_BilletPole_SwerveOffset:2
- Flush:26: STRU_001_BilletBlock:3 ↔ STRU_006_BilletPole_SwerveOffset:2
- Mate:189: COTS_95615A120_Medium-Strength Steel Nylon-Insert Locknut:11 ↔ STRU_006_BilletPole_SwerveOffset:2
- Mate:190: COTS_95615A120_Medium-Strength Steel Nylon-Insert Locknut:12 ↔ STRU_006_BilletPole_SwerveOffset:2
- Mate:194: COTS_95615A120_Medium-Strength Steel Nylon-Insert Locknut:3 ↔ STRU_006_BilletPole_SwerveOffset:1
- Mate:195: COTS_95615A120_Medium-Strength Steel Nylon-Insert Locknut:4 ↔ STRU_006_BilletPole_SwerveOffset:1
- Flush:28: STRU_003_BilletPole_28in_Angled_Unique:1 ↔ STRU_012_BilletPoleMiddle:6
- Mate:221: STRU_003_BilletPole_28in_Angled_Unique:1 ↔ STRU_012_BilletPoleMiddle:6
- Flush:29: STRU_003_BilletPole_28in_Angled_Unique:1 ↔ STRU_012_BilletPoleMiddle:5
- Mate:223: STRU_003_BilletPole_28in_Angled_Unique:1 ↔ STRU_012_BilletPoleMiddle:5
- Mate:228: STRU_012_BilletPoleMiddle:6 ↔ STRU_001_BilletBlock:14
- Mate:229: STRU_012_BilletPoleMiddle:6 ↔ STRU_001_BilletBlock:14
- Flush:30: STRU_012_BilletPoleMiddle:6 ↔ STRU_001_BilletBlock:14
- Mate:230: STRU_012_BilletPoleMiddle:5 ↔ STRU_001_BilletBlock:15
- Mate:231: STRU_012_BilletPoleMiddle:5 ↔ STRU_001_BilletBlock:15
- Flush:31: STRU_012_BilletPoleMiddle:5 ↔ STRU_001_BilletBlock:15
- Mate:253: STRU_012_BilletPoleMiddle:5 ↔ STRU_014_BilletPole_9in_Angled:2
- Flush:48: STRU_012_BilletPoleMiddle:5 ↔ STRU_014_BilletPole_9in_Angled:2
- Mate:255: STRU_012_BilletPoleMiddle:6 ↔ STRU_014_BilletPole_9in_Angled:1
- Flush:49: STRU_012_BilletPoleMiddle:6 ↔ STRU_014_BilletPole_9in_Angled:1
- Mate:257: STRU_015_BilletPole_9in:1 ↔ STRU_001_BilletBlock:19
- Mate:258: STRU_015_BilletPole_9in:1 ↔ STRU_001_BilletBlock:19
- Mate:259: STRU_015_BilletPole_9in:1 ↔ STRU_001_BilletBlock:18
- Mate:260: STRU_015_BilletPole_9in:1 ↔ STRU_001_BilletBlock:18
- Flush:52: STRU_015_BilletPole_9in:1 ↔ STRU_001_BilletBlock:18
- Flush:53: STRU_015_BilletPole_9in:1 ↔ STRU_001_BilletBlock:19
- Mate:265: STRU_001_BilletBlock:19 ↔ STRU_012_BilletPoleMiddle_Unique:1
- Mate:266: STRU_001_BilletBlock:18 ↔ STRU_012_BilletPoleMiddle_Unique:2
- Mate:267: STRU_001_BilletBlock:16 ↔ STRU_012_BilletPoleMiddle_Unique:1
- Mate:268: STRU_001_BilletBlock:16 ↔ STRU_012_BilletPoleMiddle_Unique:1
- Flush:54: STRU_001_BilletBlock:16 ↔ STRU_012_BilletPoleMiddle_Unique:1
- Mate:269: STRU_001_BilletBlock:17 ↔ STRU_012_BilletPoleMiddle_Unique:2
- Mate:270: STRU_001_BilletBlock:17 ↔ STRU_012_BilletPoleMiddle_Unique:2
- Flush:55: STRU_001_BilletBlock:17 ↔ STRU_012_BilletPoleMiddle_Unique:2
- Mate:271: STRU_001_BilletBlock:18 ↔ STRU_012_BilletPoleMiddle_Unique:2
- Mate:272: STRU_001_BilletBlock:19 ↔ STRU_012_BilletPoleMiddle_Unique:1
- Mate:275: STRU_001_BilletBlock:18 ↔ COTS_90044A120_Black-Oxide Alloy Steel Socket Head Screw:13
- Mate:276: STRU_001_BilletBlock:19 ↔ COTS_90044A120_Black-Oxide Alloy Steel Socket Head Screw:14
- Mate:277: STRU_012_BilletPoleMiddle_Unique:1 ↔ STRU_016_FrameBracket2_90:1
- Mate:278: STRU_012_BilletPoleMiddle_Unique:1 ↔ STRU_016_FrameBracket2_90:1
- Mate:279: STRU_012_BilletPoleMiddle_Unique:1 ↔ STRU_016_FrameBracket2_90:1
- Mate:280: COTS_90044A120_Black-Oxide Alloy Steel Socket Head Screw:14 ↔ STRU_016_FrameBracket2_90:1
- Mate:281: STRU_012_BilletPoleMiddle_Unique:2 ↔ STRU_016_FrameBracket2_90:2
- Mate:282: STRU_012_BilletPoleMiddle_Unique:2 ↔ STRU_016_FrameBracket2_90:2
- Mate:283: STRU_012_BilletPoleMiddle_Unique:2 ↔ STRU_016_FrameBracket2_90:2
- Mate:284: COTS_90044A120_Black-Oxide Alloy Steel Socket Head Screw:13 ↔ STRU_016_FrameBracket2_90:2
- [Mate]: COTS_90044A123_Black-Oxide Alloy Steel Socket Head Screw:18 ↔ COTS_95615A120_Medium-Strength Steel Nylon-Insert Locknut:17
- Mate:286: STRU_016_FrameBracket2_90:2 ↔ COTS_90044A123_Black-Oxide Alloy Steel Socket Head Screw:18
- Mate:288: STRU_016_FrameBracket2_90:2 ↔ COTS_90044A123_Black-Oxide Alloy Steel Socket Head Screw:18
- [Mate]: COTS_90044A123_Black-Oxide Alloy Steel Socket Head Screw:19 ↔ COTS_95615A120_Medium-Strength Steel Nylon-Insert Locknut:18
- Mate:290: STRU_016_FrameBracket2_90:2 ↔ COTS_90044A123_Black-Oxide Alloy Steel Socket Head Screw:19
- Mate:291: STRU_014_BilletPole_9in_Angled:2 ↔ COTS_95615A120_Medium-Strength Steel Nylon-Insert Locknut:18
- Mate:292: STRU_016_FrameBracket2_90:2 ↔ COTS_90044A123_Black-Oxide Alloy Steel Socket Head Screw:19
- [Mate]: COTS_90044A123_Black-Oxide Alloy Steel Socket Head Screw:20 ↔ COTS_95615A120_Medium-Strength Steel Nylon-Insert Locknut:19
- Mate:294: STRU_016_FrameBracket2_90:2 ↔ COTS_90044A123_Black-Oxide Alloy Steel Socket Head Screw:20
- Mate:295: STRU_012_BilletPoleMiddle_Unique:2 ↔ COTS_95615A120_Medium-Strength Steel Nylon-Insert Locknut:19
- Mate:296: STRU_016_FrameBracket2_90:2 ↔ COTS_90044A123_Black-Oxide Alloy Steel Socket Head Screw:20
- [Mate]: COTS_90044A123_Black-Oxide Alloy Steel Socket Head Screw:21 ↔ COTS_95615A120_Medium-Strength Steel Nylon-Insert Locknut:20
- Mate:298: STRU_016_FrameBracket2_90:2 ↔ COTS_90044A123_Black-Oxide Alloy Steel Socket Head Screw:21
- Mate:299: STRU_012_BilletPoleMiddle_Unique:2 ↔ COTS_95615A120_Medium-Strength Steel Nylon-Insert Locknut:20
- Mate:300: STRU_016_FrameBracket2_90:2 ↔ COTS_90044A123_Black-Oxide Alloy Steel Socket Head Screw:21
- [Mate]: COTS_90044A123_Black-Oxide Alloy Steel Socket Head Screw:22 ↔ COTS_95615A120_Medium-Strength Steel Nylon-Insert Locknut:21
- Mate:302: STRU_016_FrameBracket2_90:1 ↔ COTS_90044A123_Black-Oxide Alloy Steel Socket Head Screw:22
- Mate:303: STRU_016_FrameBracket2_90:1 ↔ COTS_90044A123_Black-Oxide Alloy Steel Socket Head Screw:22
- Mate:304: STRU_012_BilletPoleMiddle_Unique:1 ↔ COTS_95615A120_Medium-Strength Steel Nylon-Insert Locknut:21
- [Mate]: COTS_90044A123_Black-Oxide Alloy Steel Socket Head Screw:23 ↔ COTS_95615A120_Medium-Strength Steel Nylon-Insert Locknut:22
- Mate:306: STRU_016_FrameBracket2_90:1 ↔ COTS_90044A123_Black-Oxide Alloy Steel Socket Head Screw:23
- Mate:307: STRU_016_FrameBracket2_90:1 ↔ COTS_90044A123_Black-Oxide Alloy Steel Socket Head Screw:23
- [Mate]: COTS_90044A123_Black-Oxide Alloy Steel Socket Head Screw:24 ↔ COTS_95615A120_Medium-Strength Steel Nylon-Insert Locknut:23
- Mate:310: STRU_016_FrameBracket2_90:1 ↔ COTS_90044A123_Black-Oxide Alloy Steel Socket Head Screw:24
- Mate:311: STRU_014_BilletPole_9in_Angled:1 ↔ COTS_95615A120_Medium-Strength Steel Nylon-Insert Locknut:23
- Mate:312: STRU_016_FrameBracket2_90:1 ↔ COTS_90044A123_Black-Oxide Alloy Steel Socket Head Screw:24
- [Mate]: COTS_90044A123_Black-Oxide Alloy Steel Socket Head Screw:25 ↔ COTS_95615A120_Medium-Strength Steel Nylon-Insert Locknut:24
- Mate:314: STRU_016_FrameBracket2_90:1 ↔ COTS_90044A123_Black-Oxide Alloy Steel Socket Head Screw:25
- Mate:315: STRU_016_FrameBracket2_90:1 ↔ COTS_90044A123_Black-Oxide Alloy Steel Socket Head Screw:25
- Mate:316: STRU_012_BilletPoleMiddle_Unique:1 ↔ COTS_95615A120_Medium-Strength Steel Nylon-Insert Locknut:24
- Mate:317: STRU_014_BilletPole_9in_Angled:1 ↔ STRU_017_AngleBracket_90_Plastic:1
- Mate:318: STRU_012_BilletPoleMiddle:6 ↔ STRU_017_AngleBracket_90_Plastic:1
- Mate:319: STRU_012_BilletPoleMiddle:5 ↔ STRU_017_AngleBracket_90_Plastic:2
- Mate:320: STRU_014_BilletPole_9in_Angled:2 ↔ STRU_017_AngleBracket_90_Plastic:2
- Mate:333: STRU_014_BilletPole_9in_Angled:1 ↔ COTS_91251A539_Black-Oxide Alloy Steel Socket Head Screw (1):4
- Mate:334: STRU_014_BilletPole_9in_Angled:1 ↔ COTS_91251A539_Black-Oxide Alloy Steel Socket Head Screw (1):4
- Mate:335: STRU_014_BilletPole_9in_Angled:1 ↔ COTS_91251A539_Black-Oxide Alloy Steel Socket Head Screw (1):5
- Mate:336: STRU_014_BilletPole_9in_Angled:1 ↔ COTS_91251A539_Black-Oxide Alloy Steel Socket Head Screw (1):5
- Mate:337: STRU_014_BilletPole_9in_Angled:2 ↔ COTS_91251A539_Black-Oxide Alloy Steel Socket Head Screw (1):1
- Mate:338: STRU_014_BilletPole_9in_Angled:2 ↔ COTS_91251A539_Black-Oxide Alloy Steel Socket Head Screw (1):2
- Mate:339: STRU_014_BilletPole_9in_Angled:2 ↔ COTS_91251A539_Black-Oxide Alloy Steel Socket Head Screw (1):2
- Mate:340: STRU_014_BilletPole_9in_Angled:2 ↔ COTS_91251A539_Black-Oxide Alloy Steel Socket Head Screw (1):1
- Mate:389: STRU_012_BilletPoleMiddle:6 ↔ COTS_90044A123_Black-Oxide Alloy Steel Socket Head Screw:28
- Mate:390: STRU_012_BilletPoleMiddle:6 ↔ COTS_90044A123_Black-Oxide Alloy Steel Socket Head Screw:27
- Mate:391: STRU_012_BilletPoleMiddle:5 ↔ COTS_90044A123_Black-Oxide Alloy Steel Socket Head Screw:30
- Mate:392: STRU_012_BilletPoleMiddle:5 ↔ COTS_90044A123_Black-Oxide Alloy Steel Socket Head Screw:29
- Mate:416: STRU_012_BilletPoleMiddle:5 ↔ COTS_90044A123_Black-Oxide Alloy Steel Socket Head Screw:30
- Mate:417: STRU_012_BilletPoleMiddle:5 ↔ COTS_90044A123_Black-Oxide Alloy Steel Socket Head Screw:29
- Mate:418: STRU_012_BilletPoleMiddle:6 ↔ COTS_90044A123_Black-Oxide Alloy Steel Socket Head Screw:28
- Mate:419: STRU_012_BilletPoleMiddle:6 ↔ COTS_90044A123_Black-Oxide Alloy Steel Socket Head Screw:27
- Mate:432: COTS_91251A539_Black-Oxide Alloy Steel Socket Head Screw (1):2 ↔ COTS_95462A029_Medium-Strength Steel Hex Nut (2):1
- Mate:433: COTS_91251A539_Black-Oxide Alloy Steel Socket Head Screw (1):2 ↔ STRU_019_RubberWasher:1
- Mate:434: STRU_017_AngleBracket_90_Plastic:2 ↔ STRU_019_RubberWasher:1
- Mate:435: STRU_017_AngleBracket_90_Plastic:2 ↔ STRU_019_RubberWasher:1
- Mate:436: COTS_95462A029_Medium-Strength Steel Hex Nut (2):1 ↔ STRU_019_RubberWasher:1
- [Mate]: COTS_95462A029_Medium-Strength Steel Hex Nut (2):2 ↔ STRU_019_RubberWasher:2
- Mate:438: COTS_95462A029_Medium-Strength Steel Hex Nut (2):2 ↔ STRU_019_RubberWasher:2
- Mate:439: COTS_91251A539_Black-Oxide Alloy Steel Socket Head Screw (1):1 ↔ COTS_95462A029_Medium-Strength Steel Hex Nut (2):2
- Flush:59: STRU_019_RubberWasher:1 ↔ STRU_019_RubberWasher:2
- Mate:440: STRU_017_AngleBracket_90_Plastic:2 ↔ STRU_019_RubberWasher:2
- [Mate]: COTS_95462A029_Medium-Strength Steel Hex Nut (2):3 ↔ STRU_019_RubberWasher:3
- Mate:442: COTS_90044A123_Black-Oxide Alloy Steel Socket Head Screw:30 ↔ COTS_95462A029_Medium-Strength Steel Hex Nut (2):3
- Mate:443: COTS_90044A123_Black-Oxide Alloy Steel Socket Head Screw:30 ↔ STRU_019_RubberWasher:3
- Mate:444: STRU_017_AngleBracket_90_Plastic:2 ↔ STRU_019_RubberWasher:3
- Mate:445: STRU_017_AngleBracket_90_Plastic:2 ↔ STRU_019_RubberWasher:3
- [Mate]: COTS_95462A029_Medium-Strength Steel Hex Nut (2):4 ↔ STRU_019_RubberWasher:4
- Mate:447: COTS_95462A029_Medium-Strength Steel Hex Nut (2):4 ↔ STRU_019_RubberWasher:4
- Mate:448: COTS_90044A123_Black-Oxide Alloy Steel Socket Head Screw:29 ↔ COTS_95462A029_Medium-Strength Steel Hex Nut (2):4
- Mate:449: STRU_017_AngleBracket_90_Plastic:2 ↔ STRU_019_RubberWasher:4
- Flush:60: STRU_019_RubberWasher:3 ↔ STRU_019_RubberWasher:4
- [Mate]: COTS_95462A029_Medium-Strength Steel Hex Nut (2):5 ↔ STRU_019_RubberWasher:5
- [Mate]: COTS_95462A029_Medium-Strength Steel Hex Nut (2):5 ↔ STRU_019_RubberWasher:5
- Mate:452: COTS_91251A539_Black-Oxide Alloy Steel Socket Head Screw (1):5 ↔ COTS_95462A029_Medium-Strength Steel Hex Nut (2):5
- Mate:453: STRU_017_AngleBracket_90_Plastic:1 ↔ STRU_019_RubberWasher:5
- Mate:454: STRU_017_AngleBracket_90_Plastic:1 ↔ STRU_019_RubberWasher:5
- [Mate]: COTS_95462A029_Medium-Strength Steel Hex Nut (2):6 ↔ STRU_019_RubberWasher:6
- [Mate]: COTS_95462A029_Medium-Strength Steel Hex Nut (2):6 ↔ STRU_019_RubberWasher:6
- Mate:457: COTS_91251A539_Black-Oxide Alloy Steel Socket Head Screw (1):4 ↔ COTS_95462A029_Medium-Strength Steel Hex Nut (2):6
- Mate:458: STRU_017_AngleBracket_90_Plastic:1 ↔ STRU_019_RubberWasher:6
- Flush:61: STRU_019_RubberWasher:5 ↔ STRU_019_RubberWasher:6
- [Mate]: COTS_95462A029_Medium-Strength Steel Hex Nut (2):7 ↔ STRU_019_RubberWasher:7
- [Mate]: COTS_95462A029_Medium-Strength Steel Hex Nut (2):7 ↔ STRU_019_RubberWasher:7
- Mate:461: COTS_90044A123_Black-Oxide Alloy Steel Socket Head Screw:27 ↔ COTS_95462A029_Medium-Strength Steel Hex Nut (2):7
- Mate:462: STRU_017_AngleBracket_90_Plastic:1 ↔ STRU_019_RubberWasher:7
- Mate:463: STRU_017_AngleBracket_90_Plastic:1 ↔ STRU_019_RubberWasher:7
- [Mate]: COTS_95462A029_Medium-Strength Steel Hex Nut (2):8 ↔ STRU_019_RubberWasher:8
- [Mate]: COTS_95462A029_Medium-Strength Steel Hex Nut (2):8 ↔ STRU_019_RubberWasher:8
- Mate:466: COTS_90044A123_Black-Oxide Alloy Steel Socket Head Screw:28 ↔ COTS_95462A029_Medium-Strength Steel Hex Nut (2):8
- Mate:467: STRU_017_AngleBracket_90_Plastic:1 ↔ STRU_019_RubberWasher:8
- Flush:62: STRU_019_RubberWasher:7 ↔ STRU_019_RubberWasher:8
- Mate:470: STRU_002_BilletPole_20.56in_Angled:1 ↔ STRU_001_BilletBlock:22
- Mate:471: STRU_002_BilletPole_20.56in_Angled:1 ↔ STRU_001_BilletBlock:22
- Mate:472: STRU_023_Kenji_11in:1 ↔ STRU_001_BilletBlock:22
- Mate:473: STRU_023_Kenji_11in:1 ↔ STRU_001_BilletBlock:22
- Flush:63: STRU_002_BilletPole_20.56in_Angled:1 ↔ STRU_023_Kenji_11in:1
- Mate:475: STRU_006_BilletPole_SwerveOffset:2 ↔ STRU_023_Kenji_11in:1
- Mate:477: STRU_002_BilletPole_20.56in_Angled:2 ↔ STRU_001_BilletBlock:23
- Mate:478: STRU_002_BilletPole_20.56in_Angled:2 ↔ STRU_001_BilletBlock:23
- Mate:484: STRU_003_BilletPole_28in_Angled:2 ↔ STRU_024_BilletBlock2:1
- Mate:485: STRU_003_BilletPole_28in_Angled:2 ↔ STRU_024_BilletBlock2:6
- Mate:486: STRU_003_BilletPole_28in_Angled:2 ↔ STRU_024_BilletBlock2:5
- Mate:487: STRU_006_BilletPole_SwerveOffset:1 ↔ STRU_024_BilletBlock2:2
- Mate:488: STRU_006_BilletPole_SwerveOffset:2 ↔ STRU_024_BilletBlock2:3
- Mate:489: STRU_006_BilletPole_SwerveOffset:1 ↔ STRU_024_BilletBlock2:4
- Mate:490: STRU_003_BilletPole_28in_Angled:2 ↔ STRU_024_BilletBlock2:1
- Flush:65: STRU_001_BilletBlock:5 ↔ STRU_024_BilletBlock2:1
- Flush:66: STRU_001_BilletBlock:12 ↔ STRU_024_BilletBlock2:6
- Flush:67: STRU_024_BilletBlock2:5 ↔ STRU_024_BilletBlock2:6
- Flush:68: STRU_003_BilletPole_28in_Angled:2 ↔ STRU_003_BilletPole_28in_Angled_Unique:1
- Flush:69: STRU_024_BilletBlock2:2 ↔ STRU_024_BilletBlock2:5
- Mate:491: STRU_003_BilletPole_28in_Angled:2 ↔ STRU_024_BilletBlock2:5
- Mate:492: STRU_003_BilletPole_28in_Angled:2 ↔ STRU_024_BilletBlock2:2
- Mate:493: STRU_003_BilletPole_28in_Angled:2 ↔ STRU_024_BilletBlock2:6
- Mate:494: STRU_006_BilletPole_SwerveOffset:1 ↔ STRU_024_BilletBlock2:4
- Mate:495: STRU_006_BilletPole_SwerveOffset:2 ↔ STRU_024_BilletBlock2:3
- Flush:70: STRU_024_BilletBlock2:3 ↔ STRU_024_BilletBlock2:4
- Mate:497: STRU_009_FrameBracket_90:1 ↔ COTS_90357A021_Ultra-Low-Profile Socket Head Screw:1
- Mate:498: STRU_009_FrameBracket_90:1 ↔ COTS_90357A021_Ultra-Low-Profile Socket Head Screw:1
- Mate:499: STRU_009_FrameBracket_90:1 ↔ COTS_90357A018_Ultra-Low-Profile Socket Head Screw:1
- Mate:500: STRU_009_FrameBracket_90:1 ↔ COTS_90357A018_Ultra-Low-Profile Socket Head Screw:1
- Mate:501: STRU_009_FrameBracket_90:1 ↔ COTS_90357A018_Ultra-Low-Profile Socket Head Screw:2
- Mate:502: STRU_009_FrameBracket_90:1 ↔ COTS_90357A018_Ultra-Low-Profile Socket Head Screw:3
- Mate:503: STRU_009_FrameBracket_90:1 ↔ COTS_90357A018_Ultra-Low-Profile Socket Head Screw:4
- Mate:504: STRU_009_FrameBracket_90:4 ↔ COTS_90357A018_Ultra-Low-Profile Socket Head Screw:5
- Mate:505: STRU_009_FrameBracket_90:4 ↔ COTS_90357A018_Ultra-Low-Profile Socket Head Screw:6
- Mate:506: STRU_009_FrameBracket_90:4 ↔ COTS_90357A018_Ultra-Low-Profile Socket Head Screw:7
- Mate:507: STRU_009_FrameBracket_90:4 ↔ COTS_90357A018_Ultra-Low-Profile Socket Head Screw:8
- Mate:508: STRU_009_FrameBracket_90:4 ↔ COTS_90357A018_Ultra-Low-Profile Socket Head Screw:5
- Mate:509: STRU_009_FrameBracket_90:4 ↔ COTS_90357A018_Ultra-Low-Profile Socket Head Screw:6
- Mate:510: STRU_009_FrameBracket_90:4 ↔ COTS_90357A018_Ultra-Low-Profile Socket Head Screw:7
- Mate:511: STRU_009_FrameBracket_90:4 ↔ COTS_90357A018_Ultra-Low-Profile Socket Head Screw:8
- Mate:512: COTS_95615A120_Medium-Strength Steel Nylon-Insert Locknut:12 ↔ COTS_90357A018_Ultra-Low-Profile Socket Head Screw:8
- Mate:513: COTS_95615A120_Medium-Strength Steel Nylon-Insert Locknut:11 ↔ COTS_90357A018_Ultra-Low-Profile Socket Head Screw:7
- Mate:514: COTS_95615A120_Medium-Strength Steel Nylon-Insert Locknut:9 ↔ COTS_90357A018_Ultra-Low-Profile Socket Head Screw:5
- Mate:515: COTS_95615A120_Medium-Strength Steel Nylon-Insert Locknut:10 ↔ COTS_90357A018_Ultra-Low-Profile Socket Head Screw:6
- Mate:516: STRU_009_FrameBracket_90:1 ↔ COTS_90357A018_Ultra-Low-Profile Socket Head Screw:2
- Mate:517: STRU_009_FrameBracket_90:1 ↔ COTS_90357A018_Ultra-Low-Profile Socket Head Screw:4
- Mate:518: STRU_009_FrameBracket_90:1 ↔ COTS_90357A018_Ultra-Low-Profile Socket Head Screw:3
- Mate:519: COTS_95615A120_Medium-Strength Steel Nylon-Insert Locknut:3 ↔ COTS_90357A018_Ultra-Low-Profile Socket Head Screw:3
- Mate:520: COTS_95615A120_Medium-Strength Steel Nylon-Insert Locknut:4 ↔ COTS_90357A018_Ultra-Low-Profile Socket Head Screw:4
- Mate:521: COTS_95615A120_Medium-Strength Steel Nylon-Insert Locknut:2 ↔ COTS_90357A018_Ultra-Low-Profile Socket Head Screw:1
- Mate:522: COTS_95615A120_Medium-Strength Steel Nylon-Insert Locknut:1 ↔ COTS_90357A018_Ultra-Low-Profile Socket Head Screw:2
- Mate:523: STRU_009_FrameBracket_90:4 ↔ COTS_90357A021_Ultra-Low-Profile Socket Head Screw:2
- Mate:524: STRU_009_FrameBracket_90:4 ↔ COTS_90357A021_Ultra-Low-Profile Socket Head Screw:2
- Mate:525: STRU_006_BilletPole_SwerveOffset:2 ↔ COTS_91251A352_Black-Oxide Alloy Steel Socket Head:1
- Mate:526: STRU_006_BilletPole_SwerveOffset:2 ↔ COTS_91251A352_Black-Oxide Alloy Steel Socket Head:1
- Mate:527: STRU_002_BilletPole_20.56in_Angled:1 ↔ COTS_91251A352_Black-Oxide Alloy Steel Socket Head:2
- Mate:528: STRU_002_BilletPole_20.56in_Angled:1 ↔ COTS_91251A352_Black-Oxide Alloy Steel Socket Head:2
- Mate:529: STRU_006_BilletPole_SwerveOffset:1 ↔ COTS_91251A352_Black-Oxide Alloy Steel Socket Head:3
- Mate:530: STRU_006_BilletPole_SwerveOffset:1 ↔ COTS_91251A352_Black-Oxide Alloy Steel Socket Head:3
- Mate:531: STRU_002_BilletPole_20.56in_Angled:2 ↔ COTS_91251A352_Black-Oxide Alloy Steel Socket Head:4
- Mate:532: STRU_002_BilletPole_20.56in_Angled:2 ↔ COTS_91251A352_Black-Oxide Alloy Steel Socket Head:4
- Mate:533: STRU_006_BilletPole_SwerveOffset:1 ↔ STRU_023_Kenji_11in:2
- Flush:71: STRU_002_BilletPole_20.56in_Angled:2 ↔ STRU_023_Kenji_11in:2
- Mate:534: STRU_023_Kenji_11in:2 ↔ STRU_001_BilletBlock:23
- Mate:537: STRU_007_BilletPole_11in:1 ↔ STRU_024_BilletBlock2:1
- Mate:539: STRU_024_BilletBlock2:5 ↔ STRU_026_Bryan_11in:2
- Mate:540: STRU_024_BilletBlock2:5 ↔ STRU_026_Bryan_11in:2
- Mate:541: STRU_003_BilletPole_28in_Angled:2 ↔ STRU_026_Bryan_11in:2
- Flush:73: STRU_003_BilletPole_28in_Angled:2 ↔ STRU_026_Bryan_11in:2
- Mate:542: STRU_003_BilletPole_28in_Angled:2 ↔ COTS_90357A021_Ultra-Low-Profile Socket Head Screw:3
- Mate:543: STRU_003_BilletPole_28in_Angled:2 ↔ COTS_90357A021_Ultra-Low-Profile Socket Head Screw:3
- Mate:544: STRU_003_BilletPole_28in_Angled:2 ↔ COTS_90357A021_Ultra-Low-Profile Socket Head Screw:4
- Mate:545: STRU_003_BilletPole_28in_Angled:2 ↔ COTS_90357A021_Ultra-Low-Profile Socket Head Screw:4
- Mate:546: STRU_024_BilletBlock2:6 ↔ STRU_026_Bryan_11in:3
- Mate:547: STRU_024_BilletBlock2:6 ↔ STRU_026_Bryan_11in:3
- Flush:74: STRU_003_BilletPole_28in_Angled:2 ↔ STRU_026_Bryan_11in:3
- Mate:548: STRU_003_BilletPole_28in_Angled:2 ↔ STRU_026_Bryan_11in:3
- Mate:549: STRU_014_BilletPole_9in_Angled:1 ↔ STRU_017_AngleBracket_90_Plastic:1
- Mate:550: STRU_014_BilletPole_9in_Angled:2 ↔ STRU_017_AngleBracket_90_Plastic:2
- Mate:551: STRU_014_BilletPole_9in_Angled:1 ↔ COTS_90044A123_Black-Oxide Alloy Steel Socket Head Screw:23
- Mate:552: STRU_014_BilletPole_9in_Angled:1 ↔ COTS_90044A123_Black-Oxide Alloy Steel Socket Head Screw:24
- Mate:553: STRU_014_BilletPole_9in_Angled:2 ↔ COTS_90044A123_Black-Oxide Alloy Steel Socket Head Screw:18
- Mate:554: STRU_014_BilletPole_9in_Angled:2 ↔ COTS_90044A123_Black-Oxide Alloy Steel Socket Head Screw:19
- Mate:555: STRU_014_BilletPole_9in_Angled:2 ↔ STRU_016_FrameBracket2_90:2
- Flush:75: STRU_014_BilletPole_9in_Angled:2 ↔ STRU_015_BilletPole_9in:1
- Mate:556: STRU_014_BilletPole_9in_Angled:2 ↔ COTS_95615A120_Medium-Strength Steel Nylon-Insert Locknut:17
- Mate:557: STRU_014_BilletPole_9in_Angled:1 ↔ COTS_95615A120_Medium-Strength Steel Nylon-Insert Locknut:22
- Mate:558: STRU_014_BilletPole_9in_Angled:1 ↔ STRU_016_FrameBracket2_90:1
- Mate:559: STRU_003_BilletPole_28in_Angled_Unique:1 ↔ STRU_012_BilletPoleMiddle:6
## Named parameters: d22_d7 = 0 mm, d23_d8 = 0 mm, d24_d9 = 0 mm, d25_d10 = 0 mm, d26_d11 = 0 mm, d27_d12 = 0 mm, d389_d130 = 0 mm, d393_d130 = 0 mm, d397_d130 = 0 mm, d401_d130 = 0 mm, d405_d130 = 0 mm, d409_d130 = 0 mm, d413_d130 = 0 mm, d417_d130 = 0 mm, sa_0 = 981, sa_1 = 11120.6, sa_2 = 11120.6, sa_3 = 11120.6, sa_4 = 11120.6, d560_d559 = 0 mm, d565_d559 = 0 mm, d570_d559 = 0 mm, d575_d570_d559 = 0 mm, d576_d571 = 0 mm, d580_d575_d570_d559 = 0 mm, d581_d576_d571 = 0 mm, d585_d575_d570_d559 = 0 mm, d586_d576_d571 = 0 mm, d590_d575_d570_d559 = 0 mm, d591_d576_d571 = 0 mm
note: some values were not read from the file. Shown as the stored number, unit unknown: "sa_0", "sa_1", "sa_2", "sa_3", "sa_4".
